# Autodesk Inventor assembly: robot_with_gripper
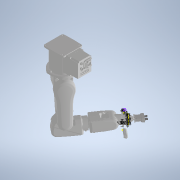
[picture p0: Inventor's stored thumbnail of the model, 180x180]
Saved by Autodesk Inventor 2021 (Build 250183000, 183)
## iProperties
Created: 2023-03-20
Part Number: robot_with_gripper
Document SubType Name: Assembly
Designer: mahmo
Author: mahmo
## Documents named in this file (3)
- D:\new_gripper\robot_with_gripper.iam
- D:\new_gripper\whole_assembly.iam
- D:\new_gripper\IRB120_3-58_irc5_rev01_step_j\IRB120_3-58_irc5_rel1_step_j\STEP Files\IRB120_3-58_IRB5_rev1_STEP_c\IRB120_3-58_IRC5_rev1.iam
## Components (2 placed, 2 different names)
1. whole_assembly:1 [sub-assembly] — Mate:1, Angle:1
2. IRB120_3-58_IRC5_rev1:1 [sub-assembly] — Mate:1, Angle:1
## Relationships (2: Mate 1, Angle 1)
- Mate:1: whole_assembly:1 ↔ IRB120_3-58_IRC5_rev1:1
- Angle:1 (0 deg): whole_assembly:1 ↔ IRB120_3-58_IRC5_rev1:1
